# Autodesk Inventor assembly: main climber
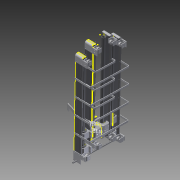
[picture p0: Inventor's stored thumbnail of the model, 180x180]
Saved by Autodesk Inventor 2013 (Build 170138000, 138)
## iProperties
Created: 2013-01-25
Part Number: main climber
Document SubType Name: Assembly
Designer: Arpan
Mass: 7886.47 g
Surface Area: 13806 cm^2
Volume: 3109.24 cm^3
Density: 2.53646 g/cm^3
Author: Arpan
## Documents named in this file (5)
- C:\Users\Moses\Documents\GitHub\frc2013CAD\Cimber actual\main climber.iam
- C:\Users\Moses\Documents\GitHub\frc2013CAD\Cimber actual\14 inch shaft.ipt
- C:\Users\Moses\Documents\GitHub\frc2013CAD\Cimber actual\Inner rails.iam
- C:\Users\Moses\Documents\GitHub\frc2013CAD\Cimber actual\outer rails.iam
- C:\Users\Moses\Documents\GitHub\frc2013CAD\Cimber actual\mini pulley assembly.iam
## Components (11 placed, 4 different names)
1. Inner rails:1 [sub-assembly] — Mate:1, Angle:1, Mate:6, Mate:7, Mate:8, Mate:9, Mate:10, Mate:11, Mate:21, Mate:22, Mate:23, Mate:24, Mate:25, Mate:26, Flush:1
2. outer rails:1 [sub-assembly] — Mate:1, Mate:2, Angle:1, Mate:3, Mate:4, Mate:5, Mate:12, Mate:13, Mate:14, Mate:15, Mate:16, Mate:17, Mate:18, Mate:19, Mate:20, Flush:1
3. 14 inch shaft:1 — Mate:2
4. mini pulley assembly:1 [sub-assembly] — Mate:3, Mate:4, Mate:5
5. mini pulley assembly:2 [sub-assembly] — Mate:6, Mate:7, Mate:8
6. mini pulley assembly:3 [sub-assembly] — Mate:24, Mate:25, Mate:26
7. mini pulley assembly:4 [sub-assembly] — Mate:9, Mate:10, Mate:11
8. mini pulley assembly:5 [sub-assembly] — Mate:18, Mate:19, Mate:20
9. mini pulley assembly:6 [sub-assembly] — Mate:12, Mate:13, Mate:14
10. mini pulley assembly:7 [sub-assembly] — Mate:15, Mate:16, Mate:17
11. mini pulley assembly:8 [sub-assembly] — Mate:21, Mate:22, Mate:23
## Relationships (28: Mate 26, Angle 1, Flush 1)
- Mate:1: Inner rails:1 ↔ outer rails:1
- Mate:2: outer rails:1 ↔ 14 inch shaft:1
- Angle:1 (180 deg): Inner rails:1 ↔ outer rails:1
- Mate:3: outer rails:1 ↔ mini pulley assembly:1
- Mate:4: outer rails:1 ↔ mini pulley assembly:1
- Mate:5: outer rails:1 ↔ mini pulley assembly:1
- Mate:6: Inner rails:1 ↔ mini pulley assembly:2
- Mate:7: Inner rails:1 ↔ mini pulley assembly:2
- Mate:8: Inner rails:1 ↔ mini pulley assembly:2
- Mate:9: Inner rails:1 ↔ mini pulley assembly:4
- Mate:10: Inner rails:1 ↔ mini pulley assembly:4
- Mate:11: Inner rails:1 ↔ mini pulley assembly:4
- Mate:12: outer rails:1 ↔ mini pulley assembly:6
- Mate:13: outer rails:1 ↔ mini pulley assembly:6
- Mate:14: outer rails:1 ↔ mini pulley assembly:6
- Mate:15: outer rails:1 ↔ mini pulley assembly:7
- Mate:16: outer rails:1 ↔ mini pulley assembly:7
- Mate:17: outer rails:1 ↔ mini pulley assembly:7
- Mate:18: outer rails:1 ↔ mini pulley assembly:5
- Mate:19: outer rails:1 ↔ mini pulley assembly:5
- Mate:20: outer rails:1 ↔ mini pulley assembly:5
- Mate:21: Inner rails:1 ↔ mini pulley assembly:8
- Mate:22: Inner rails:1 ↔ mini pulley assembly:8
- Mate:23: Inner rails:1 ↔ mini pulley assembly:8
- Mate:24: Inner rails:1 ↔ mini pulley assembly:3
- Mate:25: Inner rails:1 ↔ mini pulley assembly:3
- Mate:26: Inner rails:1 ↔ mini pulley assembly:3
- Flush:1 (12.7 mm): Inner rails:1 ↔ outer rails:1
